# Autodesk Inventor assembly: bison
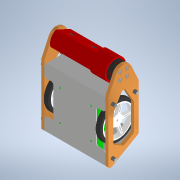
[picture p0: Inventor's stored thumbnail of the model, 180x180]
Saved by Autodesk Inventor 2021 (Build 250183000, 183)
## iProperties
Created: 2022-05-14
Part Number: bison
Document SubType Name: Assembly
Designer: ermoz
Author: ermoz
## Documents named in this file (14)
- D:\Moje Wyczyny\My_Poor_Projects\combat-bison\mechanics\bison.iam
- D:\Moje Wyczyny\My_Poor_Projects\combat-bison\mechanics\redox_bl_400_1400.ipt
- D:\Moje Wyczyny\My_Poor_Projects\combat-bison\mechanics\frame_side.ipt
- D:\Moje Wyczyny\My_Poor_Projects\combat-bison\mechanics\wheel.ipt
- D:\Moje Wyczyny\My_Poor_Projects\combat-bison\mechanics\Pololu_MicroMotor.ipt
- D:\Moje Wyczyny\My_Poor_Projects\combat-bison\mechanics\Drum.ipt
- D:\Moje Wyczyny\My_Poor_Projects\combat-bison\mechanics\battery.ipt
- D:\Moje Wyczyny\My_Poor_Projects\combat-bison\mechanics\bearing.ipt
- D:\Moje Wyczyny\My_Poor_Projects\combat-bison\mechanics\connector.ipt
- D:\Moje Wyczyny\My_Poor_Projects\combat-bison\mechanics\M3_Short_Bolt.ipt
- D:\Moje Wyczyny\My_Poor_Projects\combat-bison\mechanics\frame_side_R.ipt
- D:\Moje Wyczyny\My_Poor_Projects\combat-bison\mechanics\Pololu_MicroMotorMount.ipt
- D:\Moje Wyczyny\My_Poor_Projects\combat-bison\mechanics\armor.ipt
- D:\Moje Wyczyny\My_Poor_Projects\combat-bison\mechanics\wheel_mount.ipt
## Components (22 placed, 13 different names)
1. redox_bl_400_1400:1 — Mate:36, Mate:37, Flush:20, Mate:39, Mate:40
2. frame_side:1 — Mate:5, Mate:36, Mate:39, Mate:40, Tangent:1, Angle:1, Mate:41, Mate:42, Mate:43, Mate:44, Flush:22, Flush:23, Flush:24, Flush:25, Flush:26, Mate:45, Mate:46, Mate:53, Flush:29, Flush:31, Mate:59, Mate:62, Mate:63
3. wheel:1 — Mate:6, Mate:8, Mate:9, Mate:47
4. wheel:2 — Mate:5, Mate:6, Mate:7, Mate:10, Tangent:1
5. Pololu_MicroMotor:1 — Mate:7, Mate:10, Flush:5, Angle:1, Flush:28, Mate:51, Mate:52
6. Pololu_MicroMotor:2 — Mate:8, Mate:9, Flush:5, Mate:49, Flush:27, Mate:50
7. Drum:1 — Mate:37, Flush:20, Mate:38, Flush:21
8. battery:1 — Tangent:2, Mate:59
9. bearing:1 — Mate:38, Flush:21
10. connector:1 — Flush:31, Flush:32, Mate:55, Mate:61
11. M3_Short_Bolt:1 — Mate:41, Flush:23
12. M3_Short_Bolt:2 — Mate:44, Flush:22
13. M3_Short_Bolt:3 — Mate:43, Flush:25
14. M3_Short_Bolt:4 — Mate:42, Flush:24
15. frame_side_R:1 — Flush:26, Mate:45, Mate:46, Mate:47, Flush:30, Angle:2, Mate:58, Flush:34
16. Pololu_MicroMotorMount:1 — Flush:28, Mate:51, Mate:52, Flush:35
17. Pololu_MicroMotorMount:2 — Mate:49, Flush:27, Mate:50
18. armor:1 — Mate:53, Flush:29, Flush:30, Tangent:2
19. connector:2 — Flush:32, Flush:33, Mate:56, Mate:60, Mate:63
20. connector:3 — Flush:33, Mate:57
21. wheel_mount:1 — Mate:55, Mate:56, Angle:2, Mate:57, Mate:58, Flush:34
22. wheel_mount:2 — Mate:60, Mate:61, Mate:62, Flush:35
## Relationships (53: Mate 32, Flush 17, Tangent 2, Angle 2)
- Mate:5 (5 mm): frame_side:1 ↔ wheel:2
- Mate:6: wheel:1 ↔ wheel:2
- Mate:7: wheel:2 ↔ Pololu_MicroMotor:1
- Mate:8: wheel:1 ↔ Pololu_MicroMotor:2
- Mate:9: wheel:1 ↔ Pololu_MicroMotor:2
- Mate:10: wheel:2 ↔ Pololu_MicroMotor:1
- Flush:5: Pololu_MicroMotor:1 ↔ Pololu_MicroMotor:2
- Mate:36: redox_bl_400_1400:1 ↔ frame_side:1
- Mate:37: redox_bl_400_1400:1 ↔ Drum:1
- Flush:20: redox_bl_400_1400:1 ↔ Drum:1
- Mate:38: Drum:1 ↔ bearing:1
- Flush:21: Drum:1 ↔ bearing:1
- Mate:39: redox_bl_400_1400:1 ↔ frame_side:1
- Mate:40: redox_bl_400_1400:1 ↔ frame_side:1
- Tangent:1 (-5 mm): frame_side:1 ↔ wheel:2
- Angle:1 (0 deg): frame_side:1 ↔ Pololu_MicroMotor:1
- Mate:41: frame_side:1 ↔ M3_Short_Bolt:1
- Mate:42: frame_side:1 ↔ M3_Short_Bolt:4
- Mate:43: frame_side:1 ↔ M3_Short_Bolt:3
- Mate:44: frame_side:1 ↔ M3_Short_Bolt:2
- Flush:22: frame_side:1 ↔ M3_Short_Bolt:2
- Flush:23: frame_side:1 ↔ M3_Short_Bolt:1
- Flush:24: frame_side:1 ↔ M3_Short_Bolt:4
- Flush:25: frame_side:1 ↔ M3_Short_Bolt:3
- Flush:26: frame_side:1 ↔ frame_side_R:1
- Mate:45: frame_side:1 ↔ frame_side_R:1
- Mate:46 (100 mm): frame_side:1 ↔ frame_side_R:1
- Mate:47 (5 mm): wheel:1 ↔ frame_side_R:1
- Mate:49: Pololu_MicroMotor:2 ↔ Pololu_MicroMotorMount:2
- Flush:27: Pololu_MicroMotor:2 ↔ Pololu_MicroMotorMount:2
- Mate:50: Pololu_MicroMotor:2 ↔ Pololu_MicroMotorMount:2
- Flush:28: Pololu_MicroMotor:1 ↔ Pololu_MicroMotorMount:1
- Mate:51: Pololu_MicroMotor:1 ↔ Pololu_MicroMotorMount:1
- Mate:52: Pololu_MicroMotor:1 ↔ Pololu_MicroMotorMount:1
- Mate:53: frame_side:1 ↔ armor:1
- Flush:29: frame_side:1 ↔ armor:1
- Flush:30: frame_side_R:1 ↔ armor:1
- Flush:31 (-5 mm): frame_side:1 ↔ connector:1
- Flush:32: connector:1 ↔ connector:2
- Flush:33: connector:2 ↔ connector:3
- Mate:55: connector:1 ↔ wheel_mount:1
- Mate:56: connector:2 ↔ wheel_mount:1
- Angle:2 (0 deg): frame_side_R:1 ↔ wheel_mount:1
- Mate:57: connector:3 ↔ wheel_mount:1
- Mate:58 (15 mm): frame_side_R:1 ↔ wheel_mount:1
- Flush:34 (2 mm): frame_side_R:1 ↔ wheel_mount:1
- Tangent:2: battery:1 ↔ armor:1
- Mate:59 (36 mm): frame_side:1 ↔ battery:1
- Mate:60: connector:2 ↔ wheel_mount:2
- Mate:61: connector:1 ↔ wheel_mount:2
- Mate:62 (15 mm): frame_side:1 ↔ wheel_mount:2
- Flush:35 (6 mm): Pololu_MicroMotorMount:1 ↔ wheel_mount:2
- Mate:63: frame_side:1 ↔ connector:2
